# Autodesk Inventor assembly: frontissa
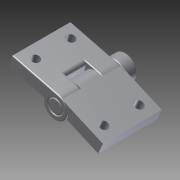
[picture p0: Inventor's stored thumbnail of the model, 180x180]
Saved by Autodesk Inventor 2012 SP1 (Build 160190100, 190)
## iProperties
Created: 2015-03-29
Part Number: frontissa
Document SubType Name: Assembly
Designer: sheina
Author: sheina
## Documents named in this file (4)
- C:\Users\Laser router cnc\Desktop\compartir con principal\impresora juan marc albert\Ultima modificacio Impresora\modificacio chasis 1-9-14\frontissa.iam
- C:\Users\Laser router cnc\Desktop\compartir con principal\impresora juan marc albert\Ultima modificacio Impresora\modificacio chasis 1-9-14\frontissa porta part1.ipt
- C:\Users\Laser router cnc\Desktop\compartir con principal\impresora juan marc albert\Ultima modificacio Impresora\modificacio chasis 1-9-14\frontissa porta part2.ipt
- C:\Users\Laser router cnc\Desktop\compartir con principal\impresora juan marc albert\Ultima modificacio Impresora\modificacio chasis 1-9-14\pern frontissa.ipt
## Components (3 placed, 3 different names)
1. frontissa porta part1:1 — Insertar:1
2. frontissa porta part2:1 — Insertar:1, Insertar:2
3. pern frontissa:1 — Insertar:2
## Relationships (2: Insert 2)
- Insertar:1: frontissa porta part1:1 ↔ frontissa porta part2:1
- Insertar:2: frontissa porta part2:1 ↔ pern frontissa:1
